# Autodesk Inventor assembly: Gripper
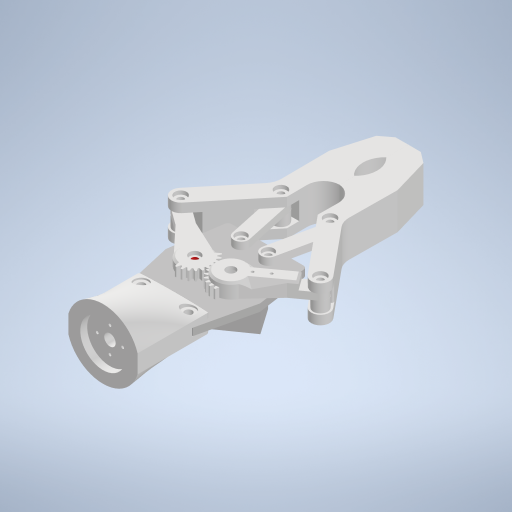
[picture p0: Inventor's stored thumbnail of the model, 512x512]
Saved by Autodesk Inventor 2023 (Build 270158000, 158)
## iProperties
Created: 2024-07-25
Part Number: Gripper
Document SubType Name: Assembly
Designer: Swoby
Author: Swoby
## Documents named in this file (9)
- C:\Users\Swoby\OneDrive\Plocha\DUM-E\V0.3\NewGripper\Gripper.iam
- C:\Users\Swoby\OneDrive\Plocha\DUM-E\V0.3\NewGripper\Claw_L.ipt
- C:\Users\Swoby\OneDrive\Plocha\DUM-E\V0.3\NewGripper\Claw_R.ipt
- C:\Users\Swoby\OneDrive\Plocha\DUM-E\V0.3\NewGripper\head.ipt
- C:\Users\Swoby\OneDrive\Plocha\DUM-E\V0.3\NewGripper\head_2.ipt
- C:\Users\Swoby\OneDrive\Plocha\DUM-E\V0.3\NewGripper\mechanism_1L.ipt
- C:\Users\Swoby\OneDrive\Plocha\DUM-E\V0.3\NewGripper\mechanism_1R.ipt
- C:\Users\Swoby\OneDrive\Plocha\DUM-E\V0.3\NewGripper\mechanism_2.ipt
- C:\Users\Swoby\OneDrive\Plocha\DUM-E\V0.3\NewGripper\vymezovak.ipt
## Components (12 placed, 8 different names)
1. Claw_L:1 — Mate:15, Mate:16, Mate:20
2. Claw_R:1 — Mate:12, Mate:13, Mate:18, Mate:25, Mate:27
3. head:1 — Mate:1, Mate:2, Mate:3, Mate:4, Mate:5, Mate:6, Mate:7, Mate:8, Mate:9, Mate:17, Mate:19
4. head_2:1 — Mate:1, Mate:2, Mate:3
5. mechanism_1L:1 — Mate:5, Mate:6, Mate:15, Mate:16, Mate:21, Mate:22
6. mechanism_1R:1 — Mate:4, Mate:7, Mate:12, Mate:13, Mate:26
7. mechanism_2:1 — Mate:8, Mate:19, Mate:20, Mate:23, Mate:24
8. mechanism_2:2 — Mate:9, Mate:17, Mate:18, Mate:28
9. vymezovak:1 — Mate:27, Mate:28
10. vymezovak:2 — Mate:25, Mate:26
11. vymezovak:3 — Mate:23, Mate:24
12. vymezovak:4 — Mate:21, Mate:22
## Relationships (25: Mate 25)
- Mate:1: head:1 ↔ head_2:1
- Mate:2: head:1 ↔ head_2:1
- Mate:3: head:1 ↔ head_2:1
- Mate:4: head:1 ↔ mechanism_1R:1
- Mate:5: head:1 ↔ mechanism_1L:1
- Mate:6: head:1 ↔ mechanism_1L:1
- Mate:7: head:1 ↔ mechanism_1R:1
- Mate:8: head:1 ↔ mechanism_2:1
- Mate:9: head:1 ↔ mechanism_2:2
- Mate:12: Claw_R:1 ↔ mechanism_1R:1
- Mate:13: Claw_R:1 ↔ mechanism_1R:1
- Mate:15: Claw_L:1 ↔ mechanism_1L:1
- Mate:16: Claw_L:1 ↔ mechanism_1L:1
- Mate:17: head:1 ↔ mechanism_2:2
- Mate:18: Claw_R:1 ↔ mechanism_2:2
- Mate:19: head:1 ↔ mechanism_2:1
- Mate:20: Claw_L:1 ↔ mechanism_2:1
- Mate:21: mechanism_1L:1 ↔ vymezovak:4
- Mate:22: mechanism_1L:1 ↔ vymezovak:4
- Mate:23: mechanism_2:1 ↔ vymezovak:3
- Mate:24: mechanism_2:1 ↔ vymezovak:3
- Mate:25: Claw_R:1 ↔ vymezovak:2
- Mate:26: mechanism_1R:1 ↔ vymezovak:2
- Mate:27: Claw_R:1 ↔ vymezovak:1
- Mate:28: mechanism_2:2 ↔ vymezovak:1
